# Autodesk Inventor assembly: 組合檔
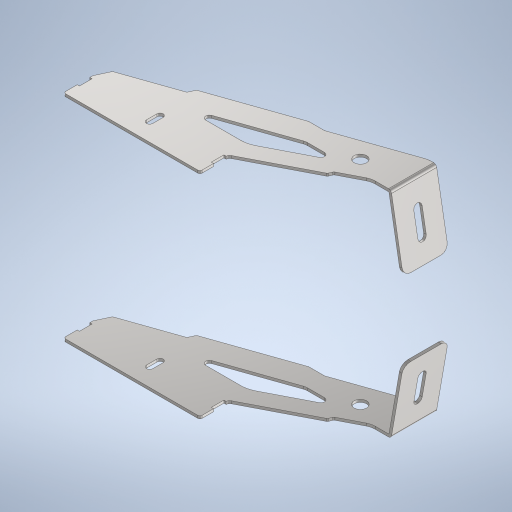
[picture p0: Inventor's stored thumbnail of the model, 512x512]
Saved by Autodesk Inventor 2023 (Build 270158000, 158)
## iProperties
Created: 2015-11-28
Part Number: 組合檔
Document SubType Name: Assembly
Designer: 設計製圖
Author: 設計製圖
## Documents named in this file (5)
- D:\資料庫\設計-工業3D\【May club 】\得利卡-車頂燈架\成品版本\生產單_22.07.14\短-車頂燈架-組合(v220714)\鏡射用--吊架-短(R)- 焊接件-1(v220714).iam
- D:\資料庫\設計-工業3D\【May club 】\得利卡-車頂燈架\成品版本\生產單_22.07.14\短-車頂燈架-組合(v220714)\吊架-短(R) - 焊接件-1(v220714).ipt
- D:\資料庫\設計-工業3D\【May club 】\得利卡-車頂燈架\成品版本\生產單_22.07.14\短-車頂燈架-組合(v220714)\吊架-短(L)- 焊接件-1_MIR(v220714).ipt
- D:\資料庫\設計-工業3D\【May club 】\得利卡-車頂燈架\成品版本\生產單_22.07.14\短-車頂燈架-組合(v220714)\吊架-短(R) - 焊接組合(v220714).iam
- D:\資料庫\設計-工業3D\【May club 】\得利卡-車頂燈架\成品版本\生產單_22.07.14\短-車頂燈架-組合(v220714)\吊架-短(R) - 焊接組合(v220714)_MIR.iam
## Components (4 placed, 4 different names)
1. 吊架-短(R) - 焊接件-1(v220714):1 — 齊平:1
2. 吊架-短(L)- 焊接件-1_MIR(v220714):1 — 貼合:1
3. 吊架-短(R) - 焊接組合(v220714)_MIR:1 [sub-assembly]
4. 吊架-短(R) - 焊接組合(v220714):1 [sub-assembly]
## Relationships (2: Flush 1, Mate 1)
- 齊平:1 [Flush] (100 mm): 吊架-短(R) - 焊接件-1(v220714):1
- 貼合:1 [Mate] (100 mm): 吊架-短(L)- 焊接件-1_MIR(v220714):1
